# Autodesk Inventor assembly: Jeep AND Krystal
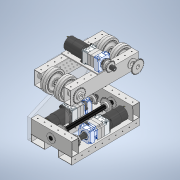
[picture p0: Inventor's stored thumbnail of the model, 180x180]
Saved by Autodesk Inventor 2020 (Build 240168000, 168)
## iProperties
Created: 2020-02-06
Part Number: Jeep AND Krystal
Document SubType Name: Assembly
Designer: aidan
Author: aidan
## Documents named in this file (3)
- C:\Users\aidan\Desktop\T3 Robotics\CAD\Jeep AND Krystal.iam
- C:\Users\aidan\Desktop\T3 Robotics\CAD\Jeep.iam
- C:\Users\aidan\Desktop\T3 Robotics\CAD\Krystal.iam
## Components (2 placed, 2 different names)
1. Jeep:1 [sub-assembly] — Mate:1
2. Krystal:1 [sub-assembly] — Mate:1
## Relationships (1: Mate 1)
- Mate:1: Jeep:1 ↔ Krystal:1
